# Autodesk Inventor assembly: 18mm-rocket-motor
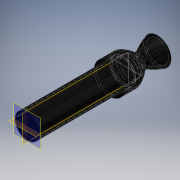
[picture p0: Inventor's stored thumbnail of the model, 180x180]
Saved by Autodesk Inventor 2017 (Build 210142000, 142)
## iProperties
Created: 2020-06-17
Part Number: 18mm-rocket-motor
Document SubType Name: Assembly
Designer: HAYNIE R&D
Author: HAYNIE R&D
## Documents named in this file (3)
- C:\Users\HAYNIE\Documents\18mm-rocket-motor\18mm-rocket-motor.iam
- C:\Users\HAYNIE\Documents\18mm-rocket-motor\motor-casing.ipt
- C:\Users\HAYNIE\Documents\18mm-rocket-motor\nozzle.ipt
## Components (2 placed, 2 different names)
1. motor-casing:1 — Rigid:1
2. nozzle:1 — Rigid:1
## Relationships (1: WeldJoint 1)
- Rigid:1 [WeldJoint] (10 mm): motor-casing:1 ↔ nozzle:1
